# Autodesk Inventor assembly: octave
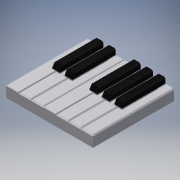
[picture p0: Inventor's stored thumbnail of the model, 180x180]
Saved by Autodesk Inventor 2017 (Build 210142000, 142)
## iProperties
Created: 2018-03-15
Part Number: octave
Document SubType Name: Assembly
Designer: Luiz Gustavo
Author: Luiz Gustavo
## Documents named in this file (5)
- C:\Users\Luiz Gustavo\Documents\Inventor\piano-robot\octave.iam
- C:\Users\Luiz Gustavo\Documents\Inventor\piano-robot\key1.ipt
- C:\Users\Luiz Gustavo\Documents\Inventor\piano-robot\key_black.ipt
- C:\Users\Luiz Gustavo\Documents\Inventor\piano-robot\key_3.ipt
- C:\Users\Luiz Gustavo\Documents\Inventor\piano-robot\key_2.ipt
## Components (12 placed, 4 different names)
1. key1:1 — Mate:1, Mate:2, Angle:1, Mate:4, Mate:6
2. key_black:1 — Mate:3, Angle:2, Mate:4
3. key_3:1 — Mate:5, Mate:6, Angle:3, Mate:8, Mate:10
4. key_2:1 — Mate:7, Mate:8, Angle:4, Mate:11
5. key_black:2 — Mate:9, Mate:10, Angle:5
6. key1:2 — Mate:11, Mate:12, Mate:15, Angle:6, Mate:22
7. key_3:2 — Mate:12, Mate:13, Mate:16, Angle:7, Mate:23
8. key_3:3 — Mate:13, Mate:14, Mate:17, Angle:8, Mate:24
9. key_2:2 — Mate:14, Mate:18, Angle:9
10. key_black:3 — Mate:19, Mate:23, Angle:11
11. key_black:4 — Mate:20, Mate:22, Angle:10
12. key_black:5 — Mate:21, Mate:24, Angle:12
## Relationships (36: Mate 24, Angle 12)
- Mate:1: key1:1
- Mate:2: key1:1
- Angle:1 (0 deg): key1:1
- Mate:3: key_black:1
- Angle:2 (180 deg): key_black:1
- Mate:4: key1:1 ↔ key_black:1
- Mate:5: key_3:1
- Mate:6: key1:1 ↔ key_3:1
- Angle:3 (0 deg): key_3:1
- Mate:7: key_2:1
- Mate:8: key_3:1 ↔ key_2:1
- Angle:4 (0 deg): key_2:1
- Mate:9: key_black:2
- Mate:10: key_3:1 ↔ key_black:2
- Angle:5 (180 deg): key_black:2
- Mate:11: key_2:1 ↔ key1:2
- Mate:12: key1:2 ↔ key_3:2
- Mate:13: key_3:2 ↔ key_3:3
- Mate:14: key_3:3 ↔ key_2:2
- Mate:15: key1:2
- Mate:16: key_3:2
- Mate:17: key_3:3
- Mate:18: key_2:2
- Angle:6 (0 deg): key1:2
- Angle:7 (0 deg): key_3:2
- Angle:8 (0 deg): key_3:3
- Angle:9 (0 deg): key_2:2
- Mate:19: key_black:3
- Mate:20: key_black:4
- Mate:21: key_black:5
- Mate:22: key1:2 ↔ key_black:4
- Mate:23: key_3:2 ↔ key_black:3
- Mate:24: key_3:3 ↔ key_black:5
- Angle:10 (180 deg): key_black:4
- Angle:11 (180 deg): key_black:3
- Angle:12 (180 deg): key_black:5
## Named parameters: maxangle = 5 deg
